# Autodesk Inventor assembly: Braille Cell
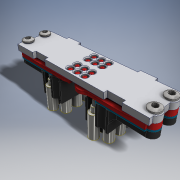
[picture p0: Inventor's stored thumbnail of the model, 180x180]
Saved by Autodesk Inventor 2016 (Build 200138000, 138)
## iProperties
Created: 2016-04-08
Part Number: Braille Cell
Document SubType Name: Assembly
Designer: Vijay
Author: Vijay
## Documents named in this file (8)
- C:\Users\Vijay\Dropbox\Personal\Braille Cell\Braille Cell.iam
- C:\Users\Vijay\Dropbox\Personal\Braille Cell\Vibration Motor.ipt
- C:\Users\Vijay\Dropbox\Personal\Braille Cell\Braille cell.ipt
- C:\Users\Vijay\Dropbox\Personal\Braille Cell\Cam.ipt
- C:\Users\Vijay\Dropbox\Personal\Braille Cell\Level1.ipt
- C:\Users\Vijay\Dropbox\Personal\Braille Cell\motor holders.ipt
- C:\Users\Vijay\Dropbox\FracktalWorks\CAD DATA\Dual Extruder Mechanism\ContentCenter\en-US\NF E 25-108 - A\NF E 25-108 - M2 x 6.ipt
- C:\Users\Vijay\Dropbox\Personal\Braille Cell\Pins_merged.ipt
## Components (35 placed, 7 different names)
1. Braille cell:1 — Mate:57, Mate:58, Mate:59, Mate:60, Angle:1, Mate:69, Mate:70
2. Vibration Motor:4 — Flush:17, Flush:20, Mate:26, Flush:25, Flush:28, Mate:71
3. Cam:1 — Mate:25, Flush:24
4. Cam:2 — Mate:26, Flush:25
5. Cam:3 — Mate:27, Flush:26
6. Level1:2 — Mate:74, Mate:75, Mate:76
7. Vibration Motor:5 — Flush:16, Flush:19, Flush:21, Flush:22, Mate:19, Mate:31, Flush:29
8. Vibration Motor:6 — Flush:14, Flush:15, Flush:19, Mate:22, Mate:27, Flush:26
9. Vibration Motor:7 — Flush:15, Flush:16, Flush:17, Flush:20, Flush:21, Mate:23, Mate:32, Flush:30
10. Vibration Motor:8 — Flush:13, Flush:18, Flush:22, Mate:21, Mate:25, Flush:24
11. Vibration Motor:9 — Flush:13, Flush:14, Flush:18, Mate:20, Mate:28, Flush:27, Flush:49
12. motor holders:1 — Mate:19, Mate:20, Mate:21, Mate:22, Mate:23, Flush:28, Angle:1, Mate:65, Mate:71, Mate:79
13. Cam:4 — Mate:28, Flush:27
14. Cam:5 — Mate:31, Flush:29
15. Cam:6 — Mate:32, Flush:30
16. Cam:7
17. Cam:8
18. Cam:9
19. Vibration Motor:10
20. Vibration Motor:11
21. Vibration Motor:12
22. Vibration Motor:13
23. Vibration Motor:14 — Flush:49
24. Vibration Motor:15
25. motor holders:2 — Mate:74, Mate:75, Mate:76, Mate:77, Mate:78
26. Cam:10
27. Cam:11
28. Cam:12
29. NF E 25-108 - A M2 x 6:1 — Mate:57, Mate:67, Mate:77
30. NF E 25-108 - A M2 x 6:2 — Mate:58, Mate:66
31. NF E 25-108 - A M2 x 6:3 — Mate:59, Mate:64
32. NF E 25-108 - A M2 x 6:4 — Mate:60, Mate:68, Mate:78
33. Level1:3 — Mate:64, Mate:65, Mate:72, Mate:79, Mate:80
34. Pins_merged:1 — Mate:67, Mate:68, Flush:63
35. Pins_merged:2 — Mate:66, Mate:69, Flush:63, Mate:70, Mate:72, Mate:80
## Relationships (80: Mate 43, Flush 36, Angle 1)
- Flush:13: Vibration Motor:8 ↔ Vibration Motor:9
- Flush:14: Vibration Motor:6 ↔ Vibration Motor:9
- Flush:15: Vibration Motor:6 ↔ Vibration Motor:7
- Flush:16: Vibration Motor:5 ↔ Vibration Motor:7
- Flush:17: Vibration Motor:4 ↔ Vibration Motor:7
- Flush:18: Vibration Motor:8 ↔ Vibration Motor:9
- Flush:19: Vibration Motor:5 ↔ Vibration Motor:6
- Flush:20: Vibration Motor:4 ↔ Vibration Motor:7
- Flush:21: Vibration Motor:5 ↔ Vibration Motor:7
- Flush:22: Vibration Motor:5 ↔ Vibration Motor:8
- Mate:19: Vibration Motor:5 ↔ motor holders:1
- Mate:20: Vibration Motor:9 ↔ motor holders:1
- Mate:21: Vibration Motor:8 ↔ motor holders:1
- Mate:22: Vibration Motor:6 ↔ motor holders:1
- Mate:23: Vibration Motor:7 ↔ motor holders:1
- Mate:25: Cam:1 ↔ Vibration Motor:8
- Mate:26: Vibration Motor:4 ↔ Cam:2
- Mate:27: Cam:3 ↔ Vibration Motor:6
- Flush:24: Cam:1 ↔ Vibration Motor:8
- Flush:25: Vibration Motor:4 ↔ Cam:2
- Flush:26: Cam:3 ↔ Vibration Motor:6
- Mate:28: Vibration Motor:9 ↔ Cam:4
- Flush:27: Vibration Motor:9 ↔ Cam:4
- Flush:28: Vibration Motor:4 ↔ motor holders:1
- Mate:31: Vibration Motor:5 ↔ Cam:5
- Mate:32: Vibration Motor:7 ↔ Cam:6
- Flush:29: Vibration Motor:5 ↔ Cam:5
- Flush:30: Vibration Motor:7 ↔ Cam:6
- [Flush]: Vibration Motor:14 ↔ Vibration Motor:15
- [Flush]: Vibration Motor:12 ↔ Vibration Motor:15
- [Flush]: Vibration Motor:12 ↔ Vibration Motor:13
- [Flush]: Vibration Motor:11 ↔ Vibration Motor:13
- [Flush]: Vibration Motor:10 ↔ Vibration Motor:13
- [Flush]: Vibration Motor:14 ↔ Vibration Motor:15
- [Flush]: Vibration Motor:11 ↔ Vibration Motor:12
- [Flush]: Vibration Motor:10 ↔ Vibration Motor:13
- [Flush]: Vibration Motor:11 ↔ Vibration Motor:13
- [Flush]: Vibration Motor:11 ↔ Vibration Motor:14
- [Mate]: Vibration Motor:11 ↔ motor holders:2
- [Mate]: Vibration Motor:15 ↔ motor holders:2
- [Mate]: Vibration Motor:14 ↔ motor holders:2
- [Mate]: Vibration Motor:12 ↔ motor holders:2
- [Mate]: Vibration Motor:13 ↔ motor holders:2
- [Mate]: Vibration Motor:10 ↔ motor holders:2
- [Mate]: Cam:7 ↔ Vibration Motor:14
- [Mate]: Cam:8 ↔ Vibration Motor:10
- [Mate]: Cam:9 ↔ Vibration Motor:12
- [Flush]: Cam:7 ↔ Vibration Motor:14
- [Flush]: Cam:8 ↔ Vibration Motor:10
- [Flush]: Cam:9 ↔ Vibration Motor:12
- [Mate]: Vibration Motor:15 ↔ Cam:10
- [Flush]: Vibration Motor:15 ↔ Cam:10
- [Flush]: Vibration Motor:10 ↔ motor holders:2
- [Mate]: Vibration Motor:11 ↔ Cam:11
- [Mate]: Vibration Motor:13 ↔ Cam:12
- [Flush]: Vibration Motor:11 ↔ Cam:11
- [Flush]: Vibration Motor:13 ↔ Cam:12
- Flush:49: Vibration Motor:9 ↔ Vibration Motor:14
- Mate:57: Braille cell:1 ↔ NF E 25-108 - A M2 x 6:1
- Mate:58: Braille cell:1 ↔ NF E 25-108 - A M2 x 6:2
- Mate:59: Braille cell:1 ↔ NF E 25-108 - A M2 x 6:3
- Mate:60: Braille cell:1 ↔ NF E 25-108 - A M2 x 6:4
- Mate:64: NF E 25-108 - A M2 x 6:3 ↔ Level1:3
- Angle:1 (0 deg): Braille cell:1 ↔ motor holders:1
- Mate:65: motor holders:1 ↔ Level1:3
- Mate:66: NF E 25-108 - A M2 x 6:2 ↔ Pins_merged:2
- Mate:67: NF E 25-108 - A M2 x 6:1 ↔ Pins_merged:1
- Mate:68: NF E 25-108 - A M2 x 6:4 ↔ Pins_merged:1
- Mate:69: Braille cell:1 ↔ Pins_merged:2
- Flush:63: Pins_merged:1 ↔ Pins_merged:2
- Mate:70: Braille cell:1 ↔ Pins_merged:2
- Mate:71: Vibration Motor:4 ↔ motor holders:1
- Mate:72: Level1:3 ↔ Pins_merged:2
- Mate:74: Level1:2 ↔ motor holders:2
- Mate:75: Level1:2 ↔ motor holders:2
- Mate:76: Level1:2 ↔ motor holders:2
- Mate:77: motor holders:2 ↔ NF E 25-108 - A M2 x 6:1
- Mate:78: motor holders:2 ↔ NF E 25-108 - A M2 x 6:4
- Mate:79: motor holders:1 ↔ Level1:3
- Mate:80: Level1:3 ↔ Pins_merged:2
## Named parameters: d74_d67 = 0 mm, d75_d70 = 0 mm, d76_d71 = 0 mm, d77_d72 = 0 mm, d78_d73 = 0 mm, d79_d61 = 0 mm, d80_d62 = 0 mm, d81_d63 = 0 mm, d82_d64 = 0 mm, d83_d65 = 0 mm, d84_d66 = 0 mm, d85_d53 = 0 mm, d86_d54 = 0 mm, d87_d55 = 0 mm, d88_d56 = 0 mm, d89_d57 = 0 mm, d90_d58 = 0 mm, d91_d59 = 0 mm, d92_d60 = 0 mm, d93_d36 = 0 mm, d94_d37 = 0 mm, d95_d38 = 0 mm, d96_d39 = 0 mm, d97_d40 = 0 mm, d98_d41 = 0 mm, d99_d42 = 0 mm, d100_d43 = 0 mm, d101_d44 = 0 mm, d102_d45 = 0 mm
